# Autodesk Inventor assembly: CardRCS
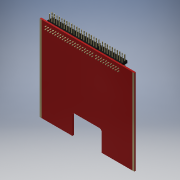
[picture p0: Inventor's stored thumbnail of the model, 180x180]
Saved by Autodesk Inventor 2017 (Build 210142000, 142)
## iProperties
Created: 2017-10-19
Part Number: CardRCS
Document SubType Name: Assembly
Designer: Bradley
Author: Bradley
## Documents named in this file (3)
- C:\Users\Bradley\Desktop\CougSat\CubeSatCardGuides\CardRCS\CardRCS.iam
- C:\Users\Bradley\Desktop\CougSat\CubeSatCardGuides\Components\CougSatBus_Male.iam
- C:\Users\Bradley\Desktop\CougSat\CubeSatCardGuides\CardRCS\CardRCS_PCB.ipt
## Components (2 placed, 2 different names)
1. CardRCS_PCB:1 — Mate:1, Mate:2, Mate:3, Mate:4
2. CougSatBus_Male:1 [sub-assembly] — Mate:1, Mate:2, Mate:3, Mate:4
## Relationships (4: Mate 4)
- Mate:1: CardRCS_PCB:1 ↔ CougSatBus_Male:1
- Mate:2 (-0.3111 mm): CardRCS_PCB:1 ↔ CougSatBus_Male:1
- Mate:3 (-0.3111 mm): CardRCS_PCB:1 ↔ CougSatBus_Male:1
- Mate:4 (-0.3111 mm): CardRCS_PCB:1 ↔ CougSatBus_Male:1
